# Autodesk Inventor assembly: robot4
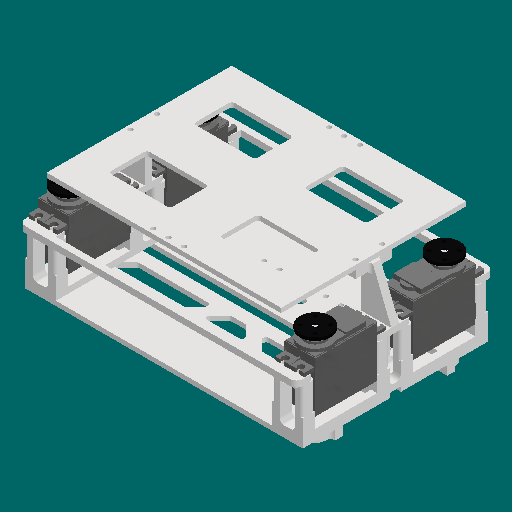
[picture p0: Inventor's stored thumbnail of the model, 512x512]
Saved by Autodesk Inventor 2026.1 (Build 301233000, 233)
## iProperties
Created: 2025-11-03
Part Number: robot4
Document SubType Name: Assembly
Designer: emanuel
Author: emanuel
## Documents named in this file (9)
- C:\Users\emanuel\UnFolder\SpiderRobo\3dmodel\body4.iam
- C:\Users\emanuel\UnFolder\SpiderRobo\3dmodel\rigid_support1.ipt
- C:\Users\emanuel\UnFolder\SpiderRobo\3dmodel\support_2_servos.ipt
- C:\Users\emanuel\UnFolder\SpiderRobo\3dmodel\mg996r.ipt
- C:\Users\emanuel\UnFolder\SpiderRobo\3dmodel\servo_support_4.ipt
- C:\Users\emanuel\UnFolder\SpiderRobo\3dmodel\rigid_support3.ipt
- C:\Users\emanuel\UnFolder\SpiderRobo\3dmodel\servo_disc.ipt
- C:\Users\emanuel\UnFolder\SpiderRobo\3dmodel\back_plate.ipt
- C:\Users\emanuel\UnFolder\SpiderRobo\3dmodel\rigid_support2.ipt
## Components (25 placed, 8 different names)
1. rigid_support1:1 — Mate:47, Mate:48, Flush:7, Flush:8, Flush:9
2. rigid_support1:2 — Flush:7, Flush:10, Flush:11, Mate:49, Flush:12, Flush:13
3. support_2_servos:3 — Mate:17, Mate:18, Mate:19, Mate:48, Mate:49, Flush:12, Flush:13, Mate:252, Flush:14, Flush:15
4. mg996r:1 — Mate:7, Mate:8, Mate:20, Mate:21, Mate:63, Mate:64, Mate:253
5. servo_support_4:3 — Flush:1, Flush:3
6. servo_support_4:4 — Flush:1, Mate:7, Mate:8, Mate:252, Flush:14, Flush:15
7. mg996r:2 — Mate:22, Mate:23, Mate:254, Mate:255
8. servo_support_4:5 — Mate:62
9. servo_support_4:6 — Flush:3, Mate:17, Mate:18, Mate:19
10. servo_disc:1 — Mate:20, Mate:21
11. servo_disc:2 — Mate:22, Mate:23
12. support_2_servos:4 — Mate:47, Flush:8, Flush:9, Flush:10, Flush:11
13. mg996r:3 — Mate:257, Mate:258
14. servo_support_4:7
15. servo_support_4:8 — Mate:256
16. rigid_support3:2 — Mate:66, Mate:67
17. mg996r:4 — Mate:260, Mate:261
18. servo_support_4:9
19. servo_support_4:10 — Mate:259
20. servo_disc:3
21. servo_disc:4
22. rigid_support3:3 — Mate:62, Mate:63, Mate:64, Mate:65, Mate:253, Mate:254, Mate:255
23. back_plate:1 — Mate:65, Mate:66, Mate:67
24. rigid_support2:1 — Mate:256, Mate:257, Mate:258
25. rigid_support2:2 — Mate:259, Mate:260, Mate:261
## Relationships (68: Mate 53, Flush 15)
- Flush:1: servo_support_4:3 ↔ servo_support_4:4
- Mate:7: mg996r:1 ↔ servo_support_4:4
- Mate:8: mg996r:1 ↔ servo_support_4:4
- [Flush]: servo_support_4:5 ↔ servo_support_4:6
- [Mate]: mg996r:2 ↔ servo_support_4:6
- [Mate]: mg996r:2 ↔ servo_support_4:6
- Flush:3: servo_support_4:3 ↔ servo_support_4:6
- Mate:17: support_2_servos:3 ↔ servo_support_4:6
- Mate:18: support_2_servos:3 ↔ servo_support_4:6
- Mate:19: support_2_servos:3 ↔ servo_support_4:6
- Mate:20: mg996r:1 ↔ servo_disc:1
- Mate:21: mg996r:1 ↔ servo_disc:1
- Mate:22: mg996r:2 ↔ servo_disc:2
- Mate:23: mg996r:2 ↔ servo_disc:2
- [Mate]: mg996r:3 ↔ rigid_support3:2
- [Mate]: mg996r:3 ↔ rigid_support3:2
- [Mate]: mg996r:3 ↔ rigid_support3:2
- [Mate]: servo_support_4:7 ↔ rigid_support3:2
- [Flush]: servo_support_4:7 ↔ servo_support_4:8
- [Mate]: servo_support_4:7 ↔ rigid_support3:2
- [Mate]: servo_support_4:7 ↔ rigid_support3:2
- [Mate]: mg996r:3 ↔ servo_support_4:8
- [Mate]: mg996r:3 ↔ servo_support_4:8
- [Flush]: servo_support_4:9 ↔ servo_support_4:10
- [Mate]: mg996r:4 ↔ servo_support_4:10
- [Mate]: mg996r:4 ↔ servo_support_4:10
- [Mate]: rigid_support3:2 ↔ servo_support_4:9
- [Mate]: rigid_support3:2 ↔ servo_support_4:9
- [Mate]: rigid_support3:2 ↔ servo_support_4:9
- [Mate]: rigid_support3:2 ↔ mg996r:4
- [Mate]: rigid_support3:2 ↔ mg996r:4
- [Mate]: rigid_support3:2 ↔ mg996r:4
- [Flush]: servo_support_4:7 ↔ servo_support_4:10
- [Mate]: support_2_servos:4 ↔ servo_support_4:10
- [Mate]: support_2_servos:4 ↔ servo_support_4:10
- [Mate]: support_2_servos:4 ↔ servo_support_4:10
- [Mate]: mg996r:3 ↔ servo_disc:3
- [Mate]: mg996r:3 ↔ servo_disc:3
- [Mate]: mg996r:4 ↔ servo_disc:4
- [Mate]: mg996r:4 ↔ servo_disc:4
- Mate:47: rigid_support1:1 ↔ support_2_servos:4
- Mate:48: rigid_support1:1 ↔ support_2_servos:3
- Flush:7: rigid_support1:1 ↔ rigid_support1:2
- Flush:8: rigid_support1:1 ↔ support_2_servos:4
- Flush:9: rigid_support1:1 ↔ support_2_servos:4
- Flush:10: rigid_support1:2 ↔ support_2_servos:4
- Flush:11: rigid_support1:2 ↔ support_2_servos:4
- Mate:49: rigid_support1:2 ↔ support_2_servos:3
- Flush:12: rigid_support1:2 ↔ support_2_servos:3
- Flush:13: rigid_support1:2 ↔ support_2_servos:3
- Mate:62: servo_support_4:5 ↔ rigid_support3:3
- Mate:63: mg996r:1 ↔ rigid_support3:3
- Mate:64: mg996r:1 ↔ rigid_support3:3
- Mate:65: rigid_support3:3 ↔ back_plate:1
- Mate:66: rigid_support3:2 ↔ back_plate:1
- Mate:67: rigid_support3:2 ↔ back_plate:1
- Mate:252: support_2_servos:3 ↔ servo_support_4:4
- Flush:14: support_2_servos:3 ↔ servo_support_4:4
- Flush:15: support_2_servos:3 ↔ servo_support_4:4
- Mate:253: mg996r:1 ↔ rigid_support3:3
- Mate:254: mg996r:2 ↔ rigid_support3:3
- Mate:255: mg996r:2 ↔ rigid_support3:3
- Mate:256: servo_support_4:8 ↔ rigid_support2:1
- Mate:257: mg996r:3 ↔ rigid_support2:1
- Mate:258: mg996r:3 ↔ rigid_support2:1
- Mate:259: servo_support_4:10 ↔ rigid_support2:2
- Mate:260: mg996r:4 ↔ rigid_support2:2
- Mate:261: mg996r:4 ↔ rigid_support2:2
## Named parameters: d24_d19 = 0 mm, d25_d22 = 0 mm, d26_d23 = 0 mm, d41_d15 = 0 mm, d42_d16 = 0 mm, d43_d17 = 0 mm, d44_d18 = 0 mm, d45_d19 = 0 mm, d46_d20 = 0 mm, d47_d21 = 0 mm, d48_d22 = 0 mm, d49_d23 = 0 mm, d50_d24_d19 = 0 mm, d51_d25_d22 = 0 mm, d52_d26_d23 = 0 mm, d53_d27 = 0 mm, d54_d28 = 0 mm, d55_d29 = 0 mm, d56_d30 = 0 mm, d57_d31 = 0 mm, d58_d32 = 0 mm, d59_d33 = 0 mm, d60_d34 = 0 mm, d61_d35 = 0 mm, d62_d36 = 0 mm, d63_d37 = 0 mm, d64_d38 = 0 mm, d65_d39 = 0 mm, d66_d40 = 0 mm
